# Autodesk Inventor assembly: UmlenkrolleHalterDoppeltAngle
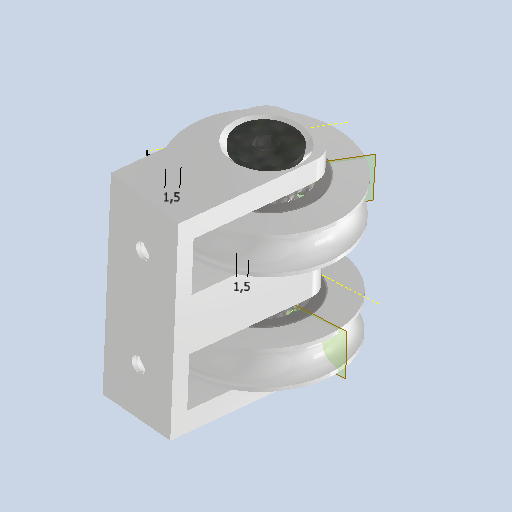
[picture p0: Inventor's stored thumbnail of the model, 512x512]
Saved by Autodesk Inventor 2025 (Build 290162010, 162A)
## iProperties
Created: 2024-11-19
Part Number: UmlenkrolleHalterDoppeltAngle
Document SubType Name: Assembly
Designer: Admin
Mass: 13.7211 g
Surface Area: 66.6118 cm^2
Volume: 4.83602 cm^3
Density: 2.83726 g/cm^3
Author: Admin
## Documents named in this file (5)
- C:\Users\Admin\GIT\HDVKBM\CAD\Krandemonstrator\UmlenkrolleHalterDoppeltAngle.iam
- C:\Users\Admin\GIT\HDVKBM\CAD\Krandemonstrator\Umlenkrolle.iam
- C:\Users\Admin\GIT\HDVKBM\CAD\Krandemonstrator\HalterUmlenkrolleDPLAngle.ipt
- C:\Users\Admin\Documents\Inventor\Content Center Files\R2025\de-DE\DIN EN ISO 7089\DIN EN ISO 7089 -  4.ipt
- C:\Users\Admin\Documents\Inventor\Content Center Files\R2025\de-DE\ISO 10642(2)\ISO 10642  - M4  x  12.ipt
## Components (9 placed, 4 different names)
1. Umlenkrolle:1 [sub-assembly] — Drehbar:9
2. DIN EN ISO 7089 4:1
3. DIN EN ISO 7089 4:2 — Drehbar:12
4. DIN EN ISO 7089 4:3 — Drehbar:9
5. Umlenkrolle:2 [sub-assembly] — Drehbar:12
6. HalterUmlenkrolleDPLAngle:1 — Starr:1, Starr:2
7. DIN EN ISO 10642 M4  x  12:1 — Starr:1
8. DIN EN ISO 10642 M4  x  12:2 — Starr:2
9. DIN EN ISO 7089 4:4
## Relationships (8: RevoluteJoint 6, WeldJoint 2)
- [RevoluteJoint]: DIN EN ISO 7089 4:3 ↔ HalterUmlenkrolleDPLAngle:1
- [RevoluteJoint]: DIN EN ISO 7089 4:2 ↔ HalterUmlenkrolleDPLAngle:1
- Drehbar:9 [RevoluteJoint]: Umlenkrolle:1 ↔ DIN EN ISO 7089 4:3
- [RevoluteJoint]: HalterUmlenkrolleDPLAngle:1 ↔ DIN EN ISO 7089 4:4
- [RevoluteJoint]: DIN EN ISO 7089 4:1 ↔ HalterUmlenkrolleDPLAngle:1
- Drehbar:12 [RevoluteJoint]: DIN EN ISO 7089 4:2 ↔ Umlenkrolle:2
- Starr:1 [WeldJoint]: HalterUmlenkrolleDPLAngle:1 ↔ DIN EN ISO 10642 M4  x  12:1
- Starr:2 [WeldJoint]: HalterUmlenkrolleDPLAngle:1 ↔ DIN EN ISO 10642 M4  x  12:2
